# Autodesk Inventor assembly: MONTAGEM_BASE_ELETRONICA
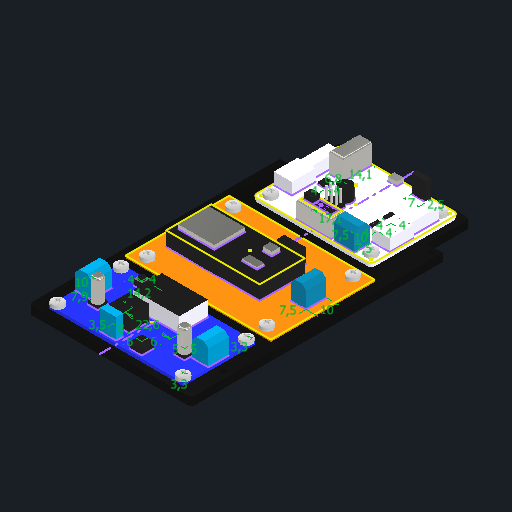
[picture p0: Inventor's stored thumbnail of the model, 512x512]
Saved by Autodesk Inventor 2027.1 (Build 311270010, 270A)
## iProperties
Created: 2026-08-16
Part Number: MONTAGEM_BASE_ELETRONICA
Document SubType Name: Assembly
Designer: Evellyn
Author: Evellyn
## Documents named in this file (6)
- C:\Users\Evellyn\Desktop\New-Robotic-Arm\mecanica\partes_ipt\MONTAGEM_BASE_ELETRONICA.iam
- C:\Users\Evellyn\Desktop\New-Robotic-Arm\mecanica\partes_ipt\BASE_ELETRONICA.ipt
- C:\Users\Evellyn\Desktop\New-Robotic-Arm\mecanica\partes_ipt\STEP_DOWN_LM2596.ipt
- C:\Users\Evellyn\Documents\Inventor\Content Center Files\R2027\pt-BR\DIN 7985 (H)\DIN 7985 (H) - M3x6-H.ipt
- C:\Users\Evellyn\Desktop\New-Robotic-Arm\mecanica\partes_ipt\PCB.ipt
- C:\Users\Evellyn\Desktop\New-Robotic-Arm\mecanica\partes_ipt\SERIAL_BUS_SERVO_CONTROLLER.ipt
## Components (16 placed, 5 different names)
1. BASE_ELETRONICA:1 — Coincidente:1, Coincidente:2, Coincidente:3, Coincidente:4, Coincidente:5, Coincidente:6, Coincidente:7, Coincidente:8, Coincidente:17, Coincidente:18, Coincidente:19, Coincidente:20, Coincidente:21, Coincidente:30, Coincidente:31, Coincidente:32, Coincidente:33, Coincidente:34
2. STEP_DOWN_LM2596:1 — Coincidente:4, Coincidente:5, Coincidente:6, Coincidente:7, Coincidente:8, Coincidente:9, Coincidente:10, Coincidente:11, Coincidente:12, Coincidente:13, Coincidente:14, Coincidente:15, Coincidente:16
3. DIN 7985 (H) M3x6-H:1 — Coincidente:9, Coincidente:10
4. DIN 7985 (H) M3x6-H:2 — Coincidente:11, Coincidente:12
5. DIN 7985 (H) M3x6-H:3 — Coincidente:13, Coincidente:14
6. DIN 7985 (H) M3x6-H:4 — Coincidente:15, Coincidente:16
7. PCB:1 — Coincidente:17, Coincidente:18, Coincidente:19, Coincidente:20, Coincidente:21, Coincidente:22, Coincidente:23, Coincidente:24, Coincidente:25, Coincidente:26, Coincidente:27, Coincidente:28, Coincidente:29
8. DIN 7985 (H) M3x6-H:5 — Coincidente:22, Coincidente:23
9. DIN 7985 (H) M3x6-H:6 — Coincidente:24, Coincidente:25
10. DIN 7985 (H) M3x6-H:7 — Coincidente:26, Coincidente:27
11. DIN 7985 (H) M3x6-H:8 — Coincidente:28, Coincidente:29
12. SERIAL_BUS_SERVO_CONTROLLER:1 — Coincidente:30, Coincidente:31, Coincidente:32, Coincidente:33, Coincidente:34, Coincidente:35, Coincidente:36, Coincidente:37, Coincidente:38, Coincidente:39, Coincidente:40, Coincidente:41, Coincidente:42
13. DIN 7985 (H) M3x6-H:9 — Coincidente:35, Coincidente:36
14. DIN 7985 (H) M3x6-H:10 — Coincidente:41, Coincidente:42
15. DIN 7985 (H) M3x6-H:11 — Coincidente:37, Coincidente:38
16. DIN 7985 (H) M3x6-H:12 — Coincidente:39, Coincidente:40
## Relationships (42: Mate 42)
- Coincidente:1 [Mate]: BASE_ELETRONICA:1
- Coincidente:2 [Mate]: BASE_ELETRONICA:1
- Coincidente:3 [Mate]: BASE_ELETRONICA:1
- Coincidente:4 [Mate]: BASE_ELETRONICA:1 ↔ STEP_DOWN_LM2596:1
- Coincidente:5 [Mate]: BASE_ELETRONICA:1 ↔ STEP_DOWN_LM2596:1
- Coincidente:6 [Mate]: BASE_ELETRONICA:1 ↔ STEP_DOWN_LM2596:1
- Coincidente:7 [Mate]: BASE_ELETRONICA:1 ↔ STEP_DOWN_LM2596:1
- Coincidente:8 [Mate]: BASE_ELETRONICA:1 ↔ STEP_DOWN_LM2596:1
- Coincidente:9 [Mate]: STEP_DOWN_LM2596:1 ↔ DIN 7985 (H) M3x6-H:1
- Coincidente:10 [Mate]: STEP_DOWN_LM2596:1 ↔ DIN 7985 (H) M3x6-H:1
- Coincidente:11 [Mate]: STEP_DOWN_LM2596:1 ↔ DIN 7985 (H) M3x6-H:2
- Coincidente:12 [Mate]: STEP_DOWN_LM2596:1 ↔ DIN 7985 (H) M3x6-H:2
- Coincidente:13 [Mate]: STEP_DOWN_LM2596:1 ↔ DIN 7985 (H) M3x6-H:3
- Coincidente:14 [Mate]: STEP_DOWN_LM2596:1 ↔ DIN 7985 (H) M3x6-H:3
- Coincidente:15 [Mate]: STEP_DOWN_LM2596:1 ↔ DIN 7985 (H) M3x6-H:4
- Coincidente:16 [Mate]: STEP_DOWN_LM2596:1 ↔ DIN 7985 (H) M3x6-H:4
- Coincidente:17 [Mate]: BASE_ELETRONICA:1 ↔ PCB:1
- Coincidente:18 [Mate]: BASE_ELETRONICA:1 ↔ PCB:1
- Coincidente:19 [Mate]: BASE_ELETRONICA:1 ↔ PCB:1
- Coincidente:20 [Mate]: BASE_ELETRONICA:1 ↔ PCB:1
- Coincidente:21 [Mate]: BASE_ELETRONICA:1 ↔ PCB:1
- Coincidente:22 [Mate]: PCB:1 ↔ DIN 7985 (H) M3x6-H:5
- Coincidente:23 [Mate]: PCB:1 ↔ DIN 7985 (H) M3x6-H:5
- Coincidente:24 [Mate]: PCB:1 ↔ DIN 7985 (H) M3x6-H:6
- Coincidente:25 [Mate]: PCB:1 ↔ DIN 7985 (H) M3x6-H:6
- Coincidente:26 [Mate]: PCB:1 ↔ DIN 7985 (H) M3x6-H:7
- Coincidente:27 [Mate]: PCB:1 ↔ DIN 7985 (H) M3x6-H:7
- Coincidente:28 [Mate]: PCB:1 ↔ DIN 7985 (H) M3x6-H:8
- Coincidente:29 [Mate]: PCB:1 ↔ DIN 7985 (H) M3x6-H:8
- Coincidente:30 [Mate]: BASE_ELETRONICA:1 ↔ SERIAL_BUS_SERVO_CONTROLLER:1
- Coincidente:31 [Mate]: BASE_ELETRONICA:1 ↔ SERIAL_BUS_SERVO_CONTROLLER:1
- Coincidente:32 [Mate]: BASE_ELETRONICA:1 ↔ SERIAL_BUS_SERVO_CONTROLLER:1
- Coincidente:33 [Mate]: BASE_ELETRONICA:1 ↔ SERIAL_BUS_SERVO_CONTROLLER:1
- Coincidente:34 [Mate]: BASE_ELETRONICA:1 ↔ SERIAL_BUS_SERVO_CONTROLLER:1
- Coincidente:35 [Mate]: SERIAL_BUS_SERVO_CONTROLLER:1 ↔ DIN 7985 (H) M3x6-H:9
- Coincidente:36 [Mate]: SERIAL_BUS_SERVO_CONTROLLER:1 ↔ DIN 7985 (H) M3x6-H:9
- Coincidente:37 [Mate]: SERIAL_BUS_SERVO_CONTROLLER:1 ↔ DIN 7985 (H) M3x6-H:11
- Coincidente:38 [Mate]: SERIAL_BUS_SERVO_CONTROLLER:1 ↔ DIN 7985 (H) M3x6-H:11
- Coincidente:39 [Mate]: SERIAL_BUS_SERVO_CONTROLLER:1 ↔ DIN 7985 (H) M3x6-H:12
- Coincidente:40 [Mate]: SERIAL_BUS_SERVO_CONTROLLER:1 ↔ DIN 7985 (H) M3x6-H:12
- Coincidente:41 [Mate]: SERIAL_BUS_SERVO_CONTROLLER:1 ↔ DIN 7985 (H) M3x6-H:10
- Coincidente:42 [Mate]: SERIAL_BUS_SERVO_CONTROLLER:1 ↔ DIN 7985 (H) M3x6-H:10
